# Autodesk Inventor assembly: LimelightCaseAssembly
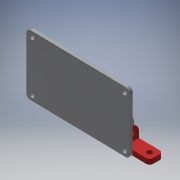
[picture p0: Inventor's stored thumbnail of the model, 180x180]
Saved by Autodesk Inventor 2018.3 (Build 223284000, 284)
## iProperties
Created: 2020-02-15
Part Number: LimelightCaseAssembly
Document SubType Name: Assembly
Designer: 22oktynich
Author: 22oktynich
## Documents named in this file (3)
- C:\Users\22oktynich\Documents\GrabCAD\Infinite Recharge 2020\Build season\Electronics\LimelightCaseAssembly.iam
- C:\Users\22oktynich\Documents\GrabCAD\Infinite Recharge 2020\Build season\Electronics\LimlightMount.ipt
- C:\Users\22oktynich\Documents\GrabCAD\Infinite Recharge 2020\Build season\Electronics\LimelightMountPivotBase.ipt
## Components (2 placed, 2 different names)
1. LimlightMount:1 — Mate:1, Mate:2
2. LimelightMountPivotBase:1 — Mate:1, Mate:2
## Relationships (2: Mate 2)
- Mate:1: LimlightMount:1 ↔ LimelightMountPivotBase:1
- Mate:2: LimlightMount:1 ↔ LimelightMountPivotBase:1
